# Autodesk Inventor assembly: Кнопки на плате
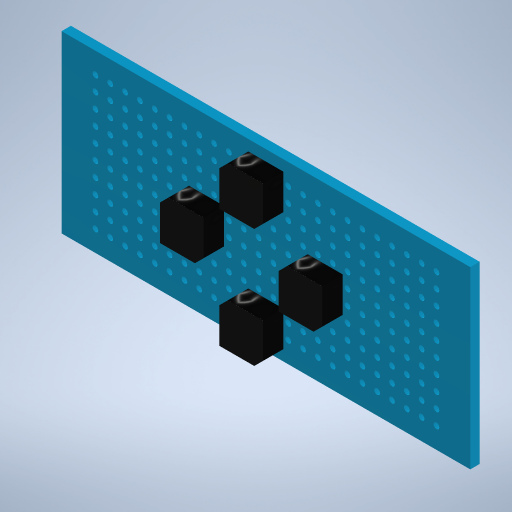
[picture p0: Inventor's stored thumbnail of the model, 512x512]
Saved by Autodesk Inventor 2024 (Build 280153020, 153B)
## iProperties
Created: 2023-06-11
Part Number: Кнопки на плате
Document SubType Name: Assembly
Designer: Admin
Author: Admin
## Documents named in this file (3)
- C:\Users\aleks\OneDrive\Рабочий стол\Хроматографический сортировщик\Детали\Покупные\Кнопки на плате.iam
- C:\Users\aleks\OneDrive\Рабочий стол\Хроматографический сортировщик\Детали\Покупные\плата панели.ipt
- C:\Users\aleks\OneDrive\Рабочий стол\Хроматографический сортировщик\Детали\Покупные\Кнопка маленькая.ipt
## Components (5 placed, 2 different names)
1. плата панели:1 — Совмещение:1, Совмещение:2, Совмещение:3, Совмещение:4, Совмещение:5, Совмещение:6, Совмещение:7, Совмещение:8, Совмещение:9
2. Кнопка маленькая:1 — Заподлицо:2, Заподлицо:3, Совмещение:1, Совмещение:2, Совмещение:3
3. Кнопка маленькая:2 — Заподлицо:3, Совмещение:8, Совмещение:9
4. Кнопка маленькая:3 — Заподлицо:1, Совмещение:4, Совмещение:5
5. Кнопка маленькая:4 — Заподлицо:1, Заподлицо:2, Совмещение:6, Совмещение:7
## Relationships (12: Mate 9, Flush 3)
- Заподлицо:1 [Flush]: Кнопка маленькая:3 ↔ Кнопка маленькая:4
- Заподлицо:2 [Flush]: Кнопка маленькая:1 ↔ Кнопка маленькая:4
- Заподлицо:3 [Flush]: Кнопка маленькая:1 ↔ Кнопка маленькая:2
- Совмещение:1 [Mate]: плата панели:1 ↔ Кнопка маленькая:1
- Совмещение:2 [Mate]: плата панели:1 ↔ Кнопка маленькая:1
- Совмещение:3 [Mate]: плата панели:1 ↔ Кнопка маленькая:1
- Совмещение:4 [Mate]: плата панели:1 ↔ Кнопка маленькая:3
- Совмещение:5 [Mate]: плата панели:1 ↔ Кнопка маленькая:3
- Совмещение:6 [Mate]: плата панели:1 ↔ Кнопка маленькая:4
- Совмещение:7 [Mate]: плата панели:1 ↔ Кнопка маленькая:4
- Совмещение:8 [Mate]: плата панели:1 ↔ Кнопка маленькая:2
- Совмещение:9 [Mate]: плата панели:1 ↔ Кнопка маленькая:2
